# Autodesk Inventor assembly: Assembly1
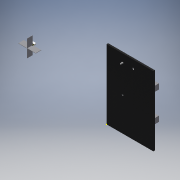
[picture p0: Inventor's stored thumbnail of the model, 180x180]
Saved by Autodesk Inventor 2019 (Build 230136000, 136)
## iProperties
Created: 2020-02-19
Part Number: Assembly1
Document SubType Name: Assembly
Designer: LENOVO
Author: LENOVO
## Documents named in this file (5)
- F:\fouzan\Assembly1.iam
- F:\fouzan\dc motor.ipt
- F:\fouzan\back plate.ipt
- F:\fouzan\servo part1.ipt
- F:\fouzan\servo part.ipt
## Components (4 placed, 4 different names)
1. dc motor:1 — Mate:1, Mate:2
2. back plate:1 — Mate:1, Mate:2
3. servo part1:1 — Mate:3, Mate:4
4. servo part:1 — Mate:3, Mate:4
## Relationships (4: Mate 4)
- Mate:1: dc motor:1 ↔ back plate:1
- Mate:2: dc motor:1 ↔ back plate:1
- Mate:3: servo part1:1 ↔ servo part:1
- Mate:4: servo part1:1 ↔ servo part:1
